# Autodesk Inventor assembly: 足ユニット
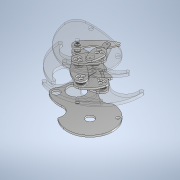
[picture p0: Inventor's stored thumbnail of the model, 180x180]
Saved by Autodesk Inventor 2022.2 (Build 262287000, 287)
## iProperties
Created: 2022-01-10
Part Number: 足ユニット
Document SubType Name: Assembly
Designer: acps
Author: acps
## Documents named in this file (4)
- C:\Users\acps\Documents\srdc\srdc_ksh\足ユニット.iam
- C:\Users\acps\Documents\srdc\srdc_ksh\足(単独).iam
- C:\Users\acps\Documents\srdc\srdc_ksh\足外フレーム.ipt
- C:\Users\acps\Documents\srdc\srdc_ksh\足内フレーム.ipt
## Components (3 placed, 3 different names)
1. 足外フレーム:1 — Insert:1, Mate:1
2. 足(単独):1 [sub-assembly] — Insert:1, Mate:1, Mate:2, Mate:3
3. 足内フレーム:1 — Mate:2, Mate:3
## Relationships (4: Mate 3, Insert 1)
- Insert:1 (0.5 mm): 足外フレーム:1 ↔ 足(単独):1
- Mate:1: 足外フレーム:1 ↔ 足(単独):1
- Mate:2: 足(単独):1 ↔ 足内フレーム:1
- Mate:3: 足(単独):1 ↔ 足内フレーム:1
